# Autodesk Inventor assembly: Gen2Plate
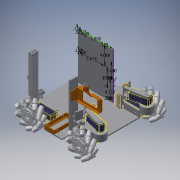
[picture p0: Inventor's stored thumbnail of the model, 180x180]
Saved by Autodesk Inventor 2017 (Build 210142000, 142)
## iProperties
Created: 2017-12-06
Part Number: Gen2Plate
Document SubType Name: Assembly
Designer: User
Author: User
## Documents named in this file (20)
- C:\Robotics\CAD\2017-18_CAD\0.1Robot.iam
- C:\Robotics\CAD\2017-18_CAD\Prototypes\Gen2PlatePart.ipt
- C:\Robotics\CAD\2017-18_CAD\Prototypes\HexMotorDirectDrive.iam
- C:\Robotics\CAD\2017-18_CAD\Prototypes\MecanumWheelFullForVexmotor.iam
- C:\Robotics\CAD\COTSParts\Rev\REV-41-1300.ipt
- C:\Robotics\CAD\2017-18_CAD\Phone_Cas.ipt
- C:\Robotics\CAD\2017-18_CAD\Prototypes\PossibleTopPlate.ipt
- C:\Robotics\CAD\2017-18_CAD\Prototypes\MotorHolderA.ipt
- C:\Robotics\CAD\2017-18_CAD\Prototypes\MotorHolderB.ipt
- C:\Robotics\CAD\2017-18_CAD\Prototypes\LeftSideTopPlateConnector.ipt
- C:\Robotics\CAD\2017-18_CAD\Prototypes\TopPlateRightConnector.ipt
- C:\Robotics\CAD\2017-18_CAD\WheelIntake5.0.iam
- C:\Robotics\CAD\2017-18_CAD\WheelIntake5.0Mirror.iam
- C:\Robotics\CAD\2017-18_CAD\WheelIntakeBrace.ipt
- C:\Robotics\CAD\2017-18_CAD\20X20lift.iam
- C:\Robotics\CAD\2017-18_CAD\WheelIntakeBraceMirror.ipt
- C:\Robotics\CAD\2017-18_CAD\GlyphLiftHolder1.ipt
- C:\Robotics\CAD\2017-18_CAD\batteryholder.ipt
- C:\Robotics\CAD\2017-18_CAD\ElectronicsPlate.ipt
- C:\Robotics\CAD\2017-18_CAD\ElectronicsPlateConnector.ipt
## Components (25 placed, 19 different names)
1. Gen2PlatePart:1 — Mate:2, Mate:8, Mate:9, Mate:10, Flush:11, Mate:11, Mate:12, Mate:13, Mate:14, Flush:14, Flush:15, Flush:16, Mate:19, Flush:18, Flush:19, Mate:49, Flush:26, Insert:1, Insert:2, Insert:5, Insert:6, Insert:9, Flush:30, Flush:31, Insert:12, Mate:57, Flush:32, Flush:33, Mate:58, Mate:60, Mate:61
2. HexMotorDirectDrive:1 [sub-assembly] — Flush:12, Mate:56, Insert:10
3. MecanumWheelFullForVexmotor:1 [sub-assembly] — Mate:6, Mate:7, Flush:12, Mate:55
4. MecanumWheelFullForVexmotor:2 [sub-assembly] — Insert:11
5. MecanumWheelFullForVexmotor:3 [sub-assembly] — Mate:15, Mate:16, Mate:54
6. REV-41-1300:2 — Mate:11, Mate:12, Mate:13, Mate:15, Mate:16, Mate:24, Mate:25, Mate:26, Mate:27, Mate:54
7. REV-41-1300:3 — Mate:6, Mate:7, Mate:8, Mate:14, Mate:20, Mate:21, Mate:22, Mate:23, Mate:55
8. REV-41-1300:4 — Mate:2, Mate:9, Mate:10, Flush:11, Mate:29, Mate:43, Mate:44, Mate:45, Insert:11
9. Phone_Cas:4 — Flush:14, Flush:15, Flush:16, Mate:37, Flush:35
10. PossibleTopPlate:1 — Mate:19, Flush:18, Flush:19, Mate:38
11. MotorHolderA:1 — Mate:24, Mate:25, Mate:26, Mate:27
12. MotorHolderA:2 — Insert:9, Flush:30, Mate:56, Insert:10, Mate:59, Flush:34
13. MotorHolderB:1 — Mate:20, Mate:21, Mate:22, Mate:23, Mate:39, Flush:21
14. MotorHolderB:2 — Mate:29, Mate:43, Mate:44, Mate:45
15. LeftSideTopPlateConnector:1 — Mate:37, Mate:60, Flush:35
16. TopPlateRightConnector:1 — Mate:38, Mate:39, Flush:21
17. WheelIntake5.0:1 [sub-assembly] — Insert:7, Insert:8
18. WheelIntake5.0Mirror:1 [sub-assembly] — Insert:3, Insert:4
19. 20X20lift:1 [sub-assembly] — Mate:49, Flush:26, Flush:31
20. WheelIntakeBrace:1 — Insert:1, Insert:2, Insert:3, Insert:4
21. WheelIntakeBraceMirror:1 — Insert:5, Insert:6, Insert:7, Insert:8
22. GlyphLiftHolder1:1 — Insert:12
23. batteryholder:2 — Mate:57, Flush:32, Flush:33
24. ElectronicsPlate:1 — Mate:58, Mate:59, Flush:34, Mate:62, Flush:36
25. ElectronicsPlateConnector:1 — Mate:61, Mate:62, Flush:36
## Relationships (66: Mate 38, Flush 16, Insert 12)
- Mate:2: Gen2PlatePart:1 ↔ REV-41-1300:4
- Mate:6: MecanumWheelFullForVexmotor:1 ↔ REV-41-1300:3
- Mate:7: MecanumWheelFullForVexmotor:1 ↔ REV-41-1300:3
- Mate:8: Gen2PlatePart:1 ↔ REV-41-1300:3
- Mate:9: Gen2PlatePart:1 ↔ REV-41-1300:4
- Mate:10: Gen2PlatePart:1 ↔ REV-41-1300:4
- Flush:11: Gen2PlatePart:1 ↔ REV-41-1300:4
- Mate:11: Gen2PlatePart:1 ↔ REV-41-1300:2
- Mate:12: Gen2PlatePart:1 ↔ REV-41-1300:2
- Mate:13: Gen2PlatePart:1 ↔ REV-41-1300:2
- Flush:12: HexMotorDirectDrive:1 ↔ MecanumWheelFullForVexmotor:1
- Mate:14: Gen2PlatePart:1 ↔ REV-41-1300:3
- Mate:15: MecanumWheelFullForVexmotor:3 ↔ REV-41-1300:2
- Mate:16: MecanumWheelFullForVexmotor:3 ↔ REV-41-1300:2
- Flush:14 (-210.7692 mm): Gen2PlatePart:1 ↔ Phone_Cas:4
- Flush:15 (-12.7 mm): Gen2PlatePart:1 ↔ Phone_Cas:4
- Flush:16: Gen2PlatePart:1 ↔ Phone_Cas:4
- Mate:19 (254 mm): Gen2PlatePart:1 ↔ PossibleTopPlate:1
- Flush:18: Gen2PlatePart:1 ↔ PossibleTopPlate:1
- Flush:19: Gen2PlatePart:1 ↔ PossibleTopPlate:1
- Mate:20: REV-41-1300:3 ↔ MotorHolderB:1
- Mate:21: REV-41-1300:3 ↔ MotorHolderB:1
- Mate:22: REV-41-1300:3 ↔ MotorHolderB:1
- Mate:23: REV-41-1300:3 ↔ MotorHolderB:1
- Mate:24: REV-41-1300:2 ↔ MotorHolderA:1
- Mate:25: REV-41-1300:2 ↔ MotorHolderA:1
- Mate:26: REV-41-1300:2 ↔ MotorHolderA:1
- Mate:27: REV-41-1300:2 ↔ MotorHolderA:1
- Mate:29: REV-41-1300:4 ↔ MotorHolderB:2
- Mate:37: Phone_Cas:4 ↔ LeftSideTopPlateConnector:1
- Mate:38: PossibleTopPlate:1 ↔ TopPlateRightConnector:1
- Mate:39: MotorHolderB:1 ↔ TopPlateRightConnector:1
- Flush:21: MotorHolderB:1 ↔ TopPlateRightConnector:1
- Mate:43: REV-41-1300:4 ↔ MotorHolderB:2
- Mate:44: REV-41-1300:4 ↔ MotorHolderB:2
- Mate:45: REV-41-1300:4 ↔ MotorHolderB:2
- Mate:49: Gen2PlatePart:1 ↔ 20X20lift:1
- Flush:26 (15.875 mm): Gen2PlatePart:1 ↔ 20X20lift:1
- Insert:1: Gen2PlatePart:1 ↔ WheelIntakeBrace:1
- Insert:2: Gen2PlatePart:1 ↔ WheelIntakeBrace:1
- Insert:3: WheelIntake5.0Mirror:1 ↔ WheelIntakeBrace:1
- Insert:4: WheelIntake5.0Mirror:1 ↔ WheelIntakeBrace:1
- Insert:5: Gen2PlatePart:1 ↔ WheelIntakeBraceMirror:1
- Insert:6: Gen2PlatePart:1 ↔ WheelIntakeBraceMirror:1
- Insert:7: WheelIntake5.0:1 ↔ WheelIntakeBraceMirror:1
- Insert:8: WheelIntake5.0:1 ↔ WheelIntakeBraceMirror:1
- Mate:54: MecanumWheelFullForVexmotor:3 ↔ REV-41-1300:2
- Mate:55: MecanumWheelFullForVexmotor:1 ↔ REV-41-1300:3
- Insert:9: Gen2PlatePart:1 ↔ MotorHolderA:2
- Flush:30: Gen2PlatePart:1 ↔ MotorHolderA:2
- Mate:56: HexMotorDirectDrive:1 ↔ MotorHolderA:2
- Insert:10: HexMotorDirectDrive:1 ↔ MotorHolderA:2
- Insert:11: MecanumWheelFullForVexmotor:2 ↔ REV-41-1300:4
- Flush:31: Gen2PlatePart:1 ↔ 20X20lift:1
- Insert:12: Gen2PlatePart:1 ↔ GlyphLiftHolder1:1
- Mate:57: Gen2PlatePart:1 ↔ batteryholder:2
- Flush:32: Gen2PlatePart:1 ↔ batteryholder:2
- Flush:33: Gen2PlatePart:1 ↔ batteryholder:2
- Mate:58: Gen2PlatePart:1 ↔ ElectronicsPlate:1
- Mate:59: MotorHolderA:2 ↔ ElectronicsPlate:1
- Flush:34 (-25.4 mm): MotorHolderA:2 ↔ ElectronicsPlate:1
- Mate:60: Gen2PlatePart:1 ↔ LeftSideTopPlateConnector:1
- Flush:35: Phone_Cas:4 ↔ LeftSideTopPlateConnector:1
- Mate:61: Gen2PlatePart:1 ↔ ElectronicsPlateConnector:1
- Mate:62: ElectronicsPlate:1 ↔ ElectronicsPlateConnector:1
- Flush:36 (-12.7 mm): ElectronicsPlate:1 ↔ ElectronicsPlateConnector:1
